# Autodesk Inventor assembly: Roller-ver3-1111-2021
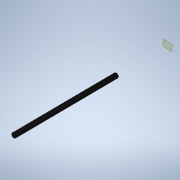
[picture p0: Inventor's stored thumbnail of the model, 180x180]
Saved by Autodesk Inventor 2021 (Build 250183000, 183)
## iProperties
Created: 2021-03-22
Part Number: Roller-ver3-1111-2021
Document SubType Name: Assembly
Designer: CMurray
Author: CMurray
## Documents named in this file (2)
- C:\Users\con_c_000\Documents\GitHub\RoboticsCad1111\PHRC CADD\2020 Infinite Recharge\Storage\Assemblies\Roller-ver3-1111-2021.iam
- C:\Users\con_c_000\Documents\GitHub\RoboticsCad1111\PHRC CADD\Resources\VEXpro Resources\Shafts\0.5inThunderHexShaft(18in)-1111-2016.ipt
## Components (1 placed, 1 different names)
1. 0.5inThunderHexShaft(18in)-1111-2016:1 — Mate:1, Angle:1
## Relationships (2: Mate 1, Angle 1)
- Mate:1: 0.5inThunderHexShaft(18in)-1111-2016:1
- Angle:1 (0 deg): 0.5inThunderHexShaft(18in)-1111-2016:1
